# Autodesk Inventor assembly: Assembly26
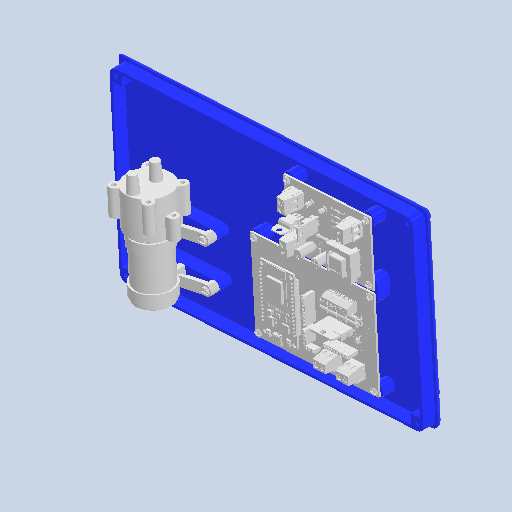
[picture p0: Inventor's stored thumbnail of the model, 512x512]
Saved by Autodesk Inventor 2024 (Build 280153000, 153)
## iProperties
Created: 2024-06-15
Part Number: Assembly26
Document SubType Name: Assembly
Designer: ASUS
Author: ASUS
## Documents named in this file (8)
- C:\Users\ASUS\Documents\Inventor\Tugas Akhir Stechoq\Assembly\Buttom Cover PCB.iam
- Assembly_Buttom_Cover.iam
- C:\Users\ASUS\Documents\Inventor\Tugas Akhir Stechoq\Part\Bottom_Cover.ipt
- C:\Users\ASUS\Documents\Inventor\Tugas Akhir Stechoq\Electronic\psustepdownFIX.ipt
- C:\Users\ASUS\Documents\Inventor\Tugas Akhir Stechoq\Electronic\SistemFix.ipt
- C:\Users\ASUS\Documents\Inventor\Tugas Akhir Stechoq\Assembly\Water Pump.iam
- C:\Users\ASUS\Documents\Inventor\Tugas Akhir Stechoq\Part\ScrewM3x0.5_PCB.ipt
- C:\Users\ASUS\Documents\Inventor\Tugas Akhir Stechoq\Part\ScrewM3.5x0.6_Motor.ipt
## Components (16 placed, 6 different names)
1. Bottom_Cover:1 — Mate:1, Mate:2, Mate:3, Mate:4, Mate:5, Mate:6, Mate:7, Mate:8, Mate:9, Mate:11, Mate:13, Mate:19, Mate:25
2. psustepdownFIX:1 — Mate:1, Mate:2, Mate:3, Mate:10, Mate:12, Mate:14, Mate:15, Mate:20, Mate:21
3. SistemFix:1 — Mate:4, Mate:5, Mate:6, Mate:16, Mate:17, Mate:18, Mate:22, Mate:23, Mate:24
4. Water Pump:1 [sub-assembly] — Mate:7, Mate:8, Mate:9, Mate:26, Mate:27, Mate:28, Mate:29, Mate:30, Mate:31, Mate:32, Mate:33
5. ScrewM3x0.5_PCB:1 — Mate:10, Mate:11
6. ScrewM3x0.5_PCB:2 — Mate:14, Mate:15
7. ScrewM3x0.5_PCB:3 — Mate:24, Mate:25
8. ScrewM3x0.5_PCB:4 — Mate:12, Mate:13
9. ScrewM3x0.5_PCB:5 — Mate:22, Mate:23
10. ScrewM3x0.5_PCB:6 — Mate:20, Mate:21
11. ScrewM3x0.5_PCB:7 — Mate:18, Mate:19
12. ScrewM3x0.5_PCB:8 — Mate:16, Mate:17
13. ScrewM3.5x0.6_Motor:1 — Mate:26, Mate:27
14. ScrewM3.5x0.6_Motor:2 — Mate:28, Mate:29
15. ScrewM3.5x0.6_Motor:3 — Mate:32, Mate:33
16. ScrewM3.5x0.6_Motor:4 — Mate:30, Mate:31
## Relationships (33: Mate 33)
- Mate:1: Bottom_Cover:1 ↔ psustepdownFIX:1
- Mate:2: Bottom_Cover:1 ↔ psustepdownFIX:1
- Mate:3: Bottom_Cover:1 ↔ psustepdownFIX:1
- Mate:4: Bottom_Cover:1 ↔ SistemFix:1
- Mate:5: Bottom_Cover:1 ↔ SistemFix:1
- Mate:6: Bottom_Cover:1 ↔ SistemFix:1
- Mate:7: Bottom_Cover:1 ↔ Water Pump:1
- Mate:8: Bottom_Cover:1 ↔ Water Pump:1
- Mate:9: Bottom_Cover:1 ↔ Water Pump:1
- Mate:10: psustepdownFIX:1 ↔ ScrewM3x0.5_PCB:1
- Mate:11: Bottom_Cover:1 ↔ ScrewM3x0.5_PCB:1
- Mate:12: psustepdownFIX:1 ↔ ScrewM3x0.5_PCB:4
- Mate:13: Bottom_Cover:1 ↔ ScrewM3x0.5_PCB:4
- Mate:14: psustepdownFIX:1 ↔ ScrewM3x0.5_PCB:2
- Mate:15: psustepdownFIX:1 ↔ ScrewM3x0.5_PCB:2
- Mate:16: SistemFix:1 ↔ ScrewM3x0.5_PCB:8
- Mate:17: SistemFix:1 ↔ ScrewM3x0.5_PCB:8
- Mate:18: SistemFix:1 ↔ ScrewM3x0.5_PCB:7
- Mate:19: Bottom_Cover:1 ↔ ScrewM3x0.5_PCB:7
- Mate:20: psustepdownFIX:1 ↔ ScrewM3x0.5_PCB:6
- Mate:21: psustepdownFIX:1 ↔ ScrewM3x0.5_PCB:6
- Mate:22: SistemFix:1 ↔ ScrewM3x0.5_PCB:5
- Mate:23: SistemFix:1 ↔ ScrewM3x0.5_PCB:5
- Mate:24: SistemFix:1 ↔ ScrewM3x0.5_PCB:3
- Mate:25: Bottom_Cover:1 ↔ ScrewM3x0.5_PCB:3
- Mate:26: Water Pump:1 ↔ ScrewM3.5x0.6_Motor:1
- Mate:27: Water Pump:1 ↔ ScrewM3.5x0.6_Motor:1
- Mate:28: Water Pump:1 ↔ ScrewM3.5x0.6_Motor:2
- Mate:29: Water Pump:1 ↔ ScrewM3.5x0.6_Motor:2
- Mate:30: Water Pump:1 ↔ ScrewM3.5x0.6_Motor:4
- Mate:31: Water Pump:1 ↔ ScrewM3.5x0.6_Motor:4
- Mate:32: Water Pump:1 ↔ ScrewM3.5x0.6_Motor:3
- Mate:33: Water Pump:1 ↔ ScrewM3.5x0.6_Motor:3
